# Autodesk Inventor assembly: am-3322+RhinoTrackDriveModule
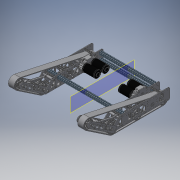
[picture p0: Inventor's stored thumbnail of the model, 180x180]
Saved by Autodesk Inventor 2016 (Build 200138000, 138)
## iProperties
Created: 2015-12-17
Part Number: am-3322+RhinoTrackDriveModule
Description: STEP AP203
Document SubType Name: Assembly
Designer: Lakhvinder
Title: am-3322 Rhino Track Drive Module.STEP
Revision Number: ANY
Sending System: SolidWorks 2014
Preprocessor: SwSTEP 2.0
## Documents named in this file (58)
- C:\Users\Lakhvinder\Desktop\Inventor Files\Andymark\am-3322+RhinoTrackDriveModule.iam
- C:\Users\Lakhvinder\Desktop\Inventor Files\Andymark\am-3319 Inside Plate.ipt
- C:\Users\Lakhvinder\Desktop\Inventor Files\Andymark\20T pulley back to back.iam
- C:\Users\Lakhvinder\Desktop\Inventor Files\Andymark\am-1393 375 washer.ipt
- C:\Users\Lakhvinder\Desktop\Inventor Files\Andymark\am-3320 Upper Bar.ipt
- C:\Users\Lakhvinder\Desktop\Inventor Files\Andymark\Track Belt.ipt
- C:\Users\Lakhvinder\Desktop\Inventor Files\Andymark\am-2598_107 2016 KOP Toughbox Mini.iam
- C:\Users\Lakhvinder\Desktop\Inventor Files\Andymark\am-3318 Outside Plate.ipt
- C:\Users\Lakhvinder\Desktop\Inventor Files\Andymark\FR8ZZ Hex Bearing.ipt
- C:\Users\Lakhvinder\Desktop\Inventor Files\Andymark\am-0207a 250 Sprocket and Pulley Spacer.ipt
- C:\Users\Lakhvinder\Desktop\Inventor Files\Andymark\10-24 Hex Washer Rolling x 1.25_93882A213.ipt
- C:\Users\Lakhvinder\Desktop\Inventor Files\Andymark\425-5M-15.ipt
- C:\Users\Lakhvinder\Desktop\Inventor Files\Andymark\500EX Hex Hub.ipt
- C:\Users\Lakhvinder\Desktop\Inventor Files\Andymark\BHCS 10-32 x 1000_SBHCSCREW 0.19-32x0.5-HX-C.ipt
- C:\Users\Lakhvinder\Desktop\Inventor Files\Andymark\10-32 Nylock Nut.ipt
- C:\Users\Lakhvinder\Desktop\Inventor Files\Andymark\0985x0420 PVC Spacer.ipt
- C:\Users\Lakhvinder\Desktop\Inventor Files\Andymark\Churro 3375.ipt
- C:\Users\Lakhvinder\Desktop\Inventor Files\Andymark\FHTS 0.25-20-0.75_FHTS 0.25-20-G-0.75-C.ipt
- C:\Users\Lakhvinder\Desktop\Inventor Files\Andymark\375-16 x 4.25 Hex Bolt_HFBOLT 0.375-16x2.5x1-C.ipt
- C:\Users\Lakhvinder\Desktop\Inventor Files\Andymark\3-8-16 NyLock Nut - Mcm 95615A140_95615A140.ipt
- C:\Users\Lakhvinder\Desktop\Inventor Files\Andymark\10-32x0625_shcs_HX-SHCS 0.19-32x1.375x1-C.ipt
- C:\Users\Lakhvinder\Desktop\Inventor Files\Andymark\187x385 spacer 13RS038518.ipt
- C:\Users\Lakhvinder\Desktop\Inventor Files\Andymark\am-0243 spacer 1860x0420.ipt
- C:\Users\Lakhvinder\Desktop\Inventor Files\Andymark\500 Hex Collar Clamp.iam
- C:\Users\Lakhvinder\Desktop\Inventor Files\Andymark\Spacer am-1181.ipt
- C:\Users\Lakhvinder\Desktop\Inventor Files\Andymark\Round Collar 375.ipt
- C:\Users\Lakhvinder\Desktop\Inventor Files\Andymark\am-2243 brass spacer.ipt
- C:\Users\Lakhvinder\Desktop\Inventor Files\Andymark\am-3321 turnbuckle.iam
- C:\Users\Lakhvinder\Desktop\Inventor Files\Andymark\am-3319 Inside Plate1.ipt
- C:\Users\Lakhvinder\Desktop\Inventor Files\Andymark\20T pulley back to back1.iam
- C:\Users\Lakhvinder\Desktop\Inventor Files\Andymark\am-1393 375 washer1.ipt
- C:\Users\Lakhvinder\Desktop\Inventor Files\Andymark\am-3320 Upper Bar1.ipt
- C:\Users\Lakhvinder\Desktop\Inventor Files\Andymark\Track Belt1.ipt
- C:\Users\Lakhvinder\Desktop\Inventor Files\Andymark\am-2598_107 2016 KOP Toughbox Mini1.iam
- C:\Users\Lakhvinder\Desktop\Inventor Files\Andymark\am-3318 Outside Plate1.ipt
- C:\Users\Lakhvinder\Desktop\Inventor Files\Andymark\FR8ZZ Hex Bearing1.ipt
- C:\Users\Lakhvinder\Desktop\Inventor Files\Andymark\am-0207a 250 Sprocket and Pulley Spacer1.ipt
- C:\Users\Lakhvinder\Desktop\Inventor Files\Andymark\10-24 Hex Washer Rolling x 1.25_93882A2131.ipt
- C:\Users\Lakhvinder\Desktop\Inventor Files\Andymark\425-5M-151.ipt
- C:\Users\Lakhvinder\Desktop\Inventor Files\Andymark\500EX Hex Hub1.ipt
- C:\Users\Lakhvinder\Desktop\Inventor Files\Andymark\BHCS 10-32 x 1000_SBHCSCREW 0.19-32x0.5-HX-C1.ipt
- C:\Users\Lakhvinder\Desktop\Inventor Files\Andymark\10-32 Nylock Nut1.ipt
- C:\Users\Lakhvinder\Desktop\Inventor Files\Andymark\0985x0420 PVC Spacer1.ipt
- C:\Users\Lakhvinder\Desktop\Inventor Files\Andymark\Churro 33751.ipt
- C:\Users\Lakhvinder\Desktop\Inventor Files\Andymark\FHTS 0.25-20-0.75_FHTS 0.25-20-G-0.75-C1.ipt
- C:\Users\Lakhvinder\Desktop\Inventor Files\Andymark\375-16 x 4.25 Hex Bolt_HFBOLT 0.375-16x2.5x1-C1.ipt
- C:\Users\Lakhvinder\Desktop\Inventor Files\Andymark\3-8-16 NyLock Nut - Mcm 95615A140_95615A1401.ipt
- C:\Users\Lakhvinder\Desktop\Inventor Files\Andymark\10-32x0625_shcs_HX-SHCS 0.19-32x1.375x1-C1.ipt
- C:\Users\Lakhvinder\Desktop\Inventor Files\Andymark\187x385 spacer 13RS0385181.ipt
- C:\Users\Lakhvinder\Desktop\Inventor Files\Andymark\am-0243 spacer 1860x04201.ipt
- C:\Users\Lakhvinder\Desktop\Inventor Files\Andymark\500 Hex Collar Clamp1.iam
- C:\Users\Lakhvinder\Desktop\Inventor Files\Andymark\Spacer am-11811.ipt
- C:\Users\Lakhvinder\Desktop\Inventor Files\Andymark\Round Collar 3751.ipt
- C:\Users\Lakhvinder\Desktop\Inventor Files\Andymark\am-2243 brass spacer1.ipt
- C:\Users\Lakhvinder\Desktop\Inventor Files\Andymark\am-3321 turnbuckle1.iam
- C:\Users\Lakhvinder\Desktop\Inventor Files\VEXpro\CIM motor.ipt
- C:\Users\Lakhvinder\Desktop\Inventor Files\VEXpro\T-Slotted Framing 20 in.ipt
- C:\Users\Lakhvinder\Desktop\Inventor Files\VEXpro\T-Slotted Framing 27.125.ipt
## Components (187 placed, 120 different names)
1. am-3319 Inside Plate_1 — Flush:1
2. 20T pulley back to back_2 [sub-assembly]
3. am-1393 375 washer_3
4. am-3320 Upper Bar_4
5. am-3320 Upper Bar_5
6. 20T pulley back to back_6 [sub-assembly]
7. Track Belt_7
8. am-2598_107 2016 KOP Toughbox Mini_8 [sub-assembly] — Mate:6, Mate:7, Mate:8, Mate:9
9. am-3318 Outside Plate_9 — Mate:16, Mate:17, Mate:18
10. 20T pulley back to back_10 [sub-assembly]
11. 20T pulley back to back_11 [sub-assembly]
12. FR8ZZ Hex Bearing_12
13. am-0207a 250 Sprocket and Pulley Spacer_13
14. 10-24 Hex Washer Rolling x 1.25_93882A213_14
15. 10-24 Hex Washer Rolling x 1.25_93882A213_15
16. 10-24 Hex Washer Rolling x 1.25_93882A213_16
17. 425-5M-15_17
18. 500EX Hex Hub_18
19. BHCS 10-32 x 1000_SBHCSCREW 0.19-32x0.5-HX-C_19
20. BHCS 10-32 x 1000_SBHCSCREW 0.19-32x0.5-HX-C_20
21. BHCS 10-32 x 1000_SBHCSCREW 0.19-32x0.5-HX-C_21
22. BHCS 10-32 x 1000_SBHCSCREW 0.19-32x0.5-HX-C_22
23. BHCS 10-32 x 1000_SBHCSCREW 0.19-32x0.5-HX-C_23
24. BHCS 10-32 x 1000_SBHCSCREW 0.19-32x0.5-HX-C_24
25. 10-32 Nylock Nut_25
26. 10-32 Nylock Nut_26
27. 10-32 Nylock Nut_27
28. 10-32 Nylock Nut_28
29. 10-32 Nylock Nut_29
30. 10-32 Nylock Nut_30
31. am-1393 375 washer_31
32. am-1393 375 washer_32
33. 0985x0420 PVC Spacer_33
34. 0985x0420 PVC Spacer_34
35. Churro 3375_35
36. Churro 3375_36
37. Churro 3375_37
38. Churro 3375_38
39. Churro 3375_39
40. Churro 3375_40
41. Churro 3375_41
42. FHTS 0.25-20-0.75_FHTS 0.25-20-G-0.75-C_42
43. FHTS 0.25-20-0.75_FHTS 0.25-20-G-0.75-C_43
44. FHTS 0.25-20-0.75_FHTS 0.25-20-G-0.75-C_44
45. FHTS 0.25-20-0.75_FHTS 0.25-20-G-0.75-C_45
46. FHTS 0.25-20-0.75_FHTS 0.25-20-G-0.75-C_46
47. FHTS 0.25-20-0.75_FHTS 0.25-20-G-0.75-C_47
48. FHTS 0.25-20-0.75_FHTS 0.25-20-G-0.75-C_48
49. FHTS 0.25-20-0.75_FHTS 0.25-20-G-0.75-C_49
50. FHTS 0.25-20-0.75_FHTS 0.25-20-G-0.75-C_50
51. FHTS 0.25-20-0.75_FHTS 0.25-20-G-0.75-C_51
52. FHTS 0.25-20-0.75_FHTS 0.25-20-G-0.75-C_52
53. FHTS 0.25-20-0.75_FHTS 0.25-20-G-0.75-C_53
54. FHTS 0.25-20-0.75_FHTS 0.25-20-G-0.75-C_54
55. FHTS 0.25-20-0.75_FHTS 0.25-20-G-0.75-C_55
56. 375-16 x 4.25 Hex Bolt_HFBOLT 0.375-16x2.5x1-C_56
57. 375-16 x 4.25 Hex Bolt_HFBOLT 0.375-16x2.5x1-C_57
58. 375-16 x 4.25 Hex Bolt_HFBOLT 0.375-16x2.5x1-C_58
59. 3-8-16 NyLock Nut - Mcm 95615A140_95615A140_59
60. 3-8-16 NyLock Nut - Mcm 95615A140_95615A140_60
61. 3-8-16 NyLock Nut - Mcm 95615A140_95615A140_61
62. 10-32x0625_shcs_HX-SHCS 0.19-32x1.375x1-C_62
63. 10-32x0625_shcs_HX-SHCS 0.19-32x1.375x1-C_63
64. 10-32x0625_shcs_HX-SHCS 0.19-32x1.375x1-C_64
65. 10-32x0625_shcs_HX-SHCS 0.19-32x1.375x1-C_65
66. FHTS 0.25-20-0.75_FHTS 0.25-20-G-0.75-C_66
67. FHTS 0.25-20-0.75_FHTS 0.25-20-G-0.75-C_67
68. FHTS 0.25-20-0.75_FHTS 0.25-20-G-0.75-C_68
69. FHTS 0.25-20-0.75_FHTS 0.25-20-G-0.75-C_69
70. am-1393 375 washer_70
71. 187x385 spacer 13RS038518_71
72. 375-16 x 4.25 Hex Bolt_HFBOLT 0.375-16x2.5x1-C_72
73. 3-8-16 NyLock Nut - Mcm 95615A140_95615A140_73
74. 3-8-16 NyLock Nut - Mcm 95615A140_95615A140_74
75. 375-16 x 4.25 Hex Bolt_HFBOLT 0.375-16x2.5x1-C_75
76. am-0243 spacer 1860x0420_76
77. am-0243 spacer 1860x0420_77
78. 500 Hex Collar Clamp_78 [sub-assembly]
79. Churro 3375_79
80. Churro 3375_80
81. 375-16 x 4.25 Hex Bolt_HFBOLT 0.375-16x2.5x1-C_81
82. 3-8-16 NyLock Nut - Mcm 95615A140_95615A140_82
83. Spacer am-1181_83
84. Round Collar 375_84
85. Round Collar 375_85
86. am-2243 brass spacer_86
87. am-2243 brass spacer_87
88. am-1393 375 washer_88
89. am-1393 375 washer_89
90. am-3321 turnbuckle_90 [sub-assembly]
91. am-3319 Inside Plate1:1 — Mate:1, Mate:10, Mate:11, Mate:12, Mate:13, Mate:14, Mate:15
92. 20T pulley back to back1:1 [sub-assembly]
93. am-1393 375 washer1:1
94. am-3320 Upper Bar1:1
95. am-3320 Upper Bar1:2
96. 20T pulley back to back1:2 [sub-assembly]
97. Track Belt1:1
98. am-2598_107 2016 KOP Toughbox Mini1:1 [sub-assembly] — Mate:2, Mate:3, Mate:4, Mate:5
99. am-3318 Outside Plate1:1
100. 20T pulley back to back1:3 [sub-assembly]
101. 20T pulley back to back1:4 [sub-assembly]
102. FR8ZZ Hex Bearing1:1
103. am-0207a 250 Sprocket and Pulley Spacer1:1
104. 10-24 Hex Washer Rolling x 1.25_93882A2131:1
105. 10-24 Hex Washer Rolling x 1.25_93882A2131:2
106. 10-24 Hex Washer Rolling x 1.25_93882A2131:3
107. 425-5M-151:1
108. 500EX Hex Hub1:1
109. BHCS 10-32 x 1000_SBHCSCREW 0.19-32x0.5-HX-C1:1
110. BHCS 10-32 x 1000_SBHCSCREW 0.19-32x0.5-HX-C1:2
111. BHCS 10-32 x 1000_SBHCSCREW 0.19-32x0.5-HX-C1:3
112. BHCS 10-32 x 1000_SBHCSCREW 0.19-32x0.5-HX-C1:4
113. BHCS 10-32 x 1000_SBHCSCREW 0.19-32x0.5-HX-C1:5
114. BHCS 10-32 x 1000_SBHCSCREW 0.19-32x0.5-HX-C1:6
115. 10-32 Nylock Nut1:1
116. 10-32 Nylock Nut1:2
117. 10-32 Nylock Nut1:3
118. 10-32 Nylock Nut1:4
119. 10-32 Nylock Nut1:5
120. 10-32 Nylock Nut1:6
121. am-1393 375 washer1:2
122. am-1393 375 washer1:3
123. 0985x0420 PVC Spacer1:1
124. 0985x0420 PVC Spacer1:2
125. Churro 33751:1
126. Churro 33751:2
127. Churro 33751:3
128. Churro 33751:4
129. Churro 33751:5
130. Churro 33751:6
131. Churro 33751:7
132. FHTS 0.25-20-0.75_FHTS 0.25-20-G-0.75-C1:1
133. FHTS 0.25-20-0.75_FHTS 0.25-20-G-0.75-C1:2
134. FHTS 0.25-20-0.75_FHTS 0.25-20-G-0.75-C1:3
135. FHTS 0.25-20-0.75_FHTS 0.25-20-G-0.75-C1:4
136. FHTS 0.25-20-0.75_FHTS 0.25-20-G-0.75-C1:5
137. FHTS 0.25-20-0.75_FHTS 0.25-20-G-0.75-C1:6
138. FHTS 0.25-20-0.75_FHTS 0.25-20-G-0.75-C1:7
139. FHTS 0.25-20-0.75_FHTS 0.25-20-G-0.75-C1:8
140. FHTS 0.25-20-0.75_FHTS 0.25-20-G-0.75-C1:9
141. FHTS 0.25-20-0.75_FHTS 0.25-20-G-0.75-C1:10
142. FHTS 0.25-20-0.75_FHTS 0.25-20-G-0.75-C1:11
143. FHTS 0.25-20-0.75_FHTS 0.25-20-G-0.75-C1:12
144. FHTS 0.25-20-0.75_FHTS 0.25-20-G-0.75-C1:13
145. FHTS 0.25-20-0.75_FHTS 0.25-20-G-0.75-C1:14
146. 375-16 x 4.25 Hex Bolt_HFBOLT 0.375-16x2.5x1-C1:1
147. 375-16 x 4.25 Hex Bolt_HFBOLT 0.375-16x2.5x1-C1:2
148. 375-16 x 4.25 Hex Bolt_HFBOLT 0.375-16x2.5x1-C1:3
149. 3-8-16 NyLock Nut - Mcm 95615A140_95615A1401:1
150. 3-8-16 NyLock Nut - Mcm 95615A140_95615A1401:2
151. 3-8-16 NyLock Nut - Mcm 95615A140_95615A1401:3
152. 10-32x0625_shcs_HX-SHCS 0.19-32x1.375x1-C1:1
153. 10-32x0625_shcs_HX-SHCS 0.19-32x1.375x1-C1:2
154. 10-32x0625_shcs_HX-SHCS 0.19-32x1.375x1-C1:3
155. 10-32x0625_shcs_HX-SHCS 0.19-32x1.375x1-C1:4
156. FHTS 0.25-20-0.75_FHTS 0.25-20-G-0.75-C1:15
157. FHTS 0.25-20-0.75_FHTS 0.25-20-G-0.75-C1:16
158. FHTS 0.25-20-0.75_FHTS 0.25-20-G-0.75-C1:17
159. FHTS 0.25-20-0.75_FHTS 0.25-20-G-0.75-C1:18
160. am-1393 375 washer1:4
161. 187x385 spacer 13RS0385181:1
162. 375-16 x 4.25 Hex Bolt_HFBOLT 0.375-16x2.5x1-C1:4
163. 3-8-16 NyLock Nut - Mcm 95615A140_95615A1401:4
164. 3-8-16 NyLock Nut - Mcm 95615A140_95615A1401:5
165. 375-16 x 4.25 Hex Bolt_HFBOLT 0.375-16x2.5x1-C1:5
166. am-0243 spacer 1860x04201:1
167. am-0243 spacer 1860x04201:2
168. 500 Hex Collar Clamp1:1 [sub-assembly]
169. Churro 33751:8
170. Churro 33751:9
171. 375-16 x 4.25 Hex Bolt_HFBOLT 0.375-16x2.5x1-C1:6
172. 3-8-16 NyLock Nut - Mcm 95615A140_95615A1401:6
173. Spacer am-11811:1
174. Round Collar 3751:1
175. Round Collar 3751:2
176. am-2243 brass spacer1:1
177. am-2243 brass spacer1:2
178. am-1393 375 washer1:5
179. am-1393 375 washer1:6
180. am-3321 turnbuckle1:1 [sub-assembly]
181. CIM motor:1 — Mate:2, Mate:3
182. CIM motor:2 — Mate:4, Mate:5
183. CIM motor:3 — Mate:7, Mate:9
184. CIM motor:4 — Mate:6, Mate:8
185. T-Slotted Framing 20 in:2 — Mate:13, Mate:14, Mate:15
186. T-Slotted Framing 20 in:3 — Mate:10, Mate:11, Mate:12
187. T-Slotted Framing 27.125:1 — Mate:16, Mate:17, Mate:18
## Relationships (19: Mate 18, Flush 1)
- Flush:1 (254 mm): am-3319 Inside Plate_1
- Mate:1 (254 mm): am-3319 Inside Plate1:1
- Mate:2: am-2598_107 2016 KOP Toughbox Mini1:1 ↔ CIM motor:1
- Mate:3: am-2598_107 2016 KOP Toughbox Mini1:1 ↔ CIM motor:1
- Mate:4: am-2598_107 2016 KOP Toughbox Mini1:1 ↔ CIM motor:2
- Mate:5: am-2598_107 2016 KOP Toughbox Mini1:1 ↔ CIM motor:2
- Mate:6: am-2598_107 2016 KOP Toughbox Mini_8 ↔ CIM motor:4
- Mate:7: am-2598_107 2016 KOP Toughbox Mini_8 ↔ CIM motor:3
- Mate:8: am-2598_107 2016 KOP Toughbox Mini_8 ↔ CIM motor:4
- Mate:9: am-2598_107 2016 KOP Toughbox Mini_8 ↔ CIM motor:3
- Mate:10: am-3319 Inside Plate1:1 ↔ T-Slotted Framing 20 in:3
- Mate:11: am-3319 Inside Plate1:1 ↔ T-Slotted Framing 20 in:3
- Mate:12: am-3319 Inside Plate1:1 ↔ T-Slotted Framing 20 in:3
- Mate:13: am-3319 Inside Plate1:1 ↔ T-Slotted Framing 20 in:2
- Mate:14: am-3319 Inside Plate1:1 ↔ T-Slotted Framing 20 in:2
- Mate:15: am-3319 Inside Plate1:1 ↔ T-Slotted Framing 20 in:2
- Mate:16: am-3318 Outside Plate_9 ↔ T-Slotted Framing 27.125:1
- Mate:17: am-3318 Outside Plate_9 ↔ T-Slotted Framing 27.125:1
- Mate:18: am-3318 Outside Plate_9 ↔ T-Slotted Framing 27.125:1
